# Autodesk Inventor assembly: Hook Whip edit
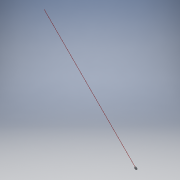
[picture p0: Inventor's stored thumbnail of the model, 180x180]
Saved by Autodesk Inventor 2016 (Build 200138000, 138)
## iProperties
Created: 2016-01-19
Part Number: Hook Whip edit
Document SubType Name: Assembly
Designer: TimB
Author: TimB
## Documents named in this file (3)
- C:\Users\TimB\Documents\GitHub\phi_robotics\3d-models\FTC_Tetrix_KOP_Block_Party\Tim Bloot Designs\JAr JaR Bot\Hook Whip edit.iam
- C:\Users\TimB\Documents\GitHub\phi_robotics\3d-models\FTC_Tetrix_KOP_Block_Party\Tetrix_Kit_FTC\Autodesk Inventor Files\tetrix_servo_horn.iam
- C:\Users\TimB\Documents\GitHub\phi_robotics\3d-models\FTC_Tetrix_KOP_Block_Party\Tim Bloot Designs\JAr JaR Bot\Hook Whip.ipt
## Components (2 placed, 2 different names)
1. tetrix_servo_horn:1 [sub-assembly] — Rigid:1
2. Hook Whip:1 — Rigid:1
## Relationships (1: WeldJoint 1)
- Rigid:1 [WeldJoint]: tetrix_servo_horn:1 ↔ Hook Whip:1
